# Autodesk Inventor assembly: 15102898-16-A-0400
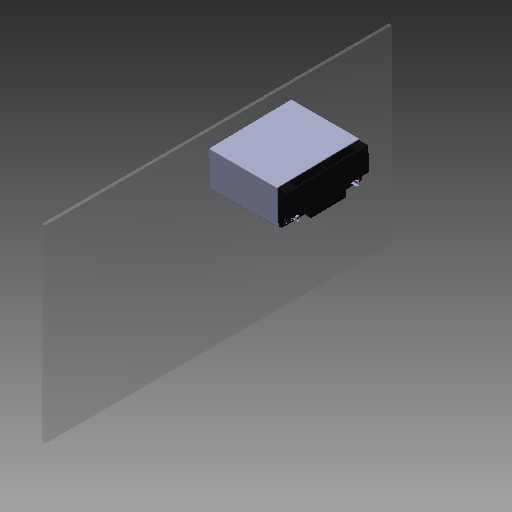
[picture p0: Inventor's stored thumbnail of the model, 512x512]
Saved by Autodesk Inventor 2017 (Build 210142000, 142)
## iProperties
Created: 2016-10-03
Part Number: 15102898-16-A-0400
Document SubType Name: Assembly
Designer: gus
Author: gus
## Documents named in this file (3)
- C:\Users\15102898\Documents\GitHub\bps-bunnybots2016-cad\Bunnybot-To_be_renamed\15102898-16-A-0000\15102898-16-A-0400\15102898-16-A-0400.iam
- C:\Users\15102898\Documents\GitHub\bps-bunnybots2016-cad\Bunnybot-To_be_renamed\15102898-16-A-0000\15102898-16-A-0400\15102898-16-P-0401.ipt
- C:\Users\15102898\Documents\GitHub\bps-bunnybots2016-cad\Bunnybot-To_be_renamed\15102898-16-A-0000\15102898-16-A-0400\Imported Components\User Library-Battery-6.ipt
## Components (2 placed, 2 different names)
1. 15102898-16-P-0401:1 — Mate:1
2. User Library-Battery-6:1 — Mate:1
## Relationships (1: Mate 1)
- Mate:1: 15102898-16-P-0401:1 ↔ User Library-Battery-6:1
